# Autodesk Inventor assembly: wheel_with_mounts
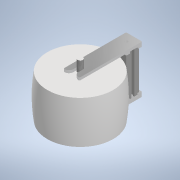
[picture p0: Inventor's stored thumbnail of the model, 180x180]
Saved by Autodesk Inventor 2021 (Build 250183000, 183)
## iProperties
Created: 2021-05-27
Part Number: wheel_with_mounts
Document SubType Name: Assembly
Designer: gisen
Author: gisen
## Documents named in this file (4)
- C:\Users\gisen\workspace\beetle_inventor_model\suspension\wheel_with_mounts.iam
- C:\Users\gisen\workspace\beetle_inventor_model\suspension\6inch_wheel.ipt
- C:\Users\gisen\workspace\beetle_inventor_model\suspension\CAM\wheel_mount.ipt
- C:\Users\gisen\workspace\beetle_inventor_model\suspension\frame\AFS-3030-97.ipt
## Components (4 placed, 3 different names)
1. 6inch_wheel:1 — メイト:1, メイト:2, メイト:3, フラッシュ:3, フラッシュ:10, メイト:12
2. wheel_mount — メイト:3, フラッシュ:3, フラッシュ:10, フラッシュ:12, メイト:12, フラッシュ:13, メイト:14, メイト:15, フラッシュ:14
3. wheel_mount:2 — メイト:13, メイト:16, フラッシュ:14
4. AFS-3030-97:1 — フラッシュ:13, メイト:13, メイト:14, メイト:15, メイト:16
## Relationships (13: Mate 8, Flush 5)
- メイト:1 [Mate]: 6inch_wheel:1
- メイト:2 [Mate]: 6inch_wheel:1
- メイト:3 [Mate]: 6inch_wheel:1 ↔ wheel_mount
- フラッシュ:3 [Flush]: 6inch_wheel:1 ↔ wheel_mount
- フラッシュ:10 [Flush]: 6inch_wheel:1 ↔ wheel_mount
- フラッシュ:12 [Flush]: wheel_mount
- メイト:12 [Mate]: 6inch_wheel:1 ↔ wheel_mount
- フラッシュ:13 [Flush]: wheel_mount ↔ AFS-3030-97:1
- メイト:13 [Mate]: wheel_mount:2 ↔ AFS-3030-97:1
- メイト:14 [Mate]: wheel_mount ↔ AFS-3030-97:1
- メイト:15 [Mate]: wheel_mount ↔ AFS-3030-97:1
- メイト:16 [Mate]: wheel_mount:2 ↔ AFS-3030-97:1
- フラッシュ:14 [Flush]: wheel_mount ↔ wheel_mount:2
